# Autodesk Inventor assembly: Mx64_with_horn_MIR_shoulder_up
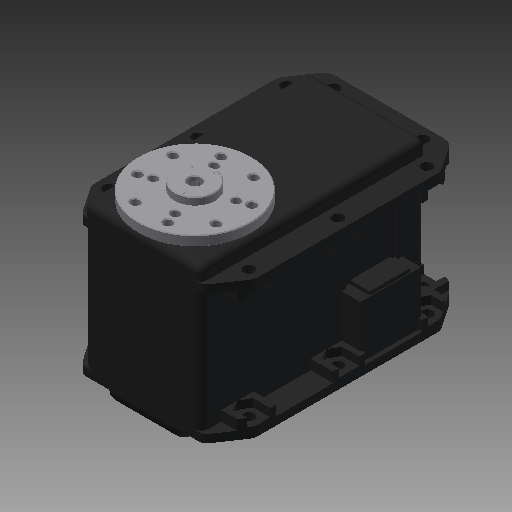
[picture p0: Inventor's stored thumbnail of the model, 512x512]
Saved by Autodesk Inventor 2019 (Build 230136000, 136)
## iProperties
Created: 2014-04-23
Part Number: Mx64_with_horn_MIR_shoulder_up
Document SubType Name: Assembly
Designer: 4wieser
Mass: 72.06 g
Surface Area: 159.232 cm^2
Volume: 72.06 cm^3
Density: 1 g/cm^3
Author: BitBots
## Documents named in this file (3)
- Z:\Nico_N\NICO-CAD-master\NICO_CAD_master\motors\Mx64\Mx64_with_horn_MIR_shoulder_up.iam
- Z:\Nico_N\NICO-CAD-master\NICO_CAD_master\motors\Mx64\MX-64T_MIR.ipt
- Z:\Nico_N\NICO-CAD-master\NICO_CAD_master\motors\HN05-N101_(mx64)\HN05-N101_MIR.ipt
## Components (2 placed, 2 different names)
1. MX-64T_MIR:1 — Rotational:1
2. HN05-N101_MIR:1 — Rotational:1
## Relationships (1: RevoluteJoint 1)
- Rotational:1 [RevoluteJoint]: MX-64T_MIR:1 ↔ HN05-N101_MIR:1
